# Autodesk Inventor assembly: DriveTrainSides
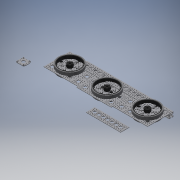
[picture p0: Inventor's stored thumbnail of the model, 180x180]
Saved by Autodesk Inventor 2018 (Build 220112000, 112)
## iProperties
Created: 2017-10-27
Part Number: DriveTrainSides
Document SubType Name: Assembly
Designer: ball
Author: ball
## Documents named in this file (6)
- C:\FTC\2017Robot\DriveTrainOutside.iam
- C:\FTC\Actobotics\585 parts\585002.ipt
- C:\FTC\Actobotics\585 parts\585724.ipt
- C:\FTC\Andymark\am-2648_4inWheel8mmHub.ipt
- C:\FTC\Actobotics\555 parts\555128.ipt
- C:\FTC\Actobotics\565 parts\565062.ipt
## Components (11 placed, 5 different names)
1. 585002:1 — Mate:5, Mate:6, Mate:10
2. 585002:2 — Mate:2, Mate:3, Mate:4
3. 585002:3 — Mate:7, Mate:8, Mate:9, Mate:11
4. 585724:1 — Mate:2, Mate:3, Mate:4, Mate:5, Mate:6
5. 585724:2 — Mate:7, Mate:8, Mate:9, Mate:10
6. am-2648_4inWheel8mmHub:1
7. am-2648_4inWheel8mmHub:2
8. am-2648_4inWheel8mmHub:3
9. 555128:1
10. 585724:3
11. 565062:1 — Mate:11
## Relationships (10: Mate 10)
- Mate:2: 585002:2 ↔ 585724:1
- Mate:3: 585002:2 ↔ 585724:1
- Mate:4: 585002:2 ↔ 585724:1
- Mate:5: 585002:1 ↔ 585724:1
- Mate:6: 585002:1 ↔ 585724:1
- Mate:7: 585002:3 ↔ 585724:2
- Mate:8: 585002:3 ↔ 585724:2
- Mate:9: 585002:3 ↔ 585724:2
- Mate:10: 585002:1 ↔ 585724:2
- Mate:11: 585002:3 ↔ 565062:1
